# Autodesk Inventor assembly: ASY DMF 01 50 tape v2.1
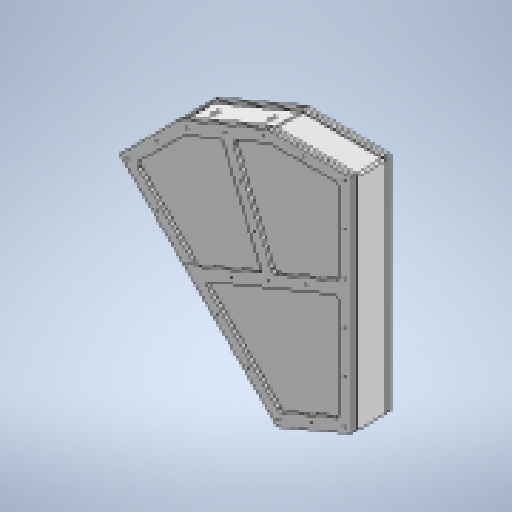
[picture p0: Inventor's stored thumbnail of the model, 512x512]
Saved by Autodesk Inventor 2025.3 (Build 293356000, 356)
## iProperties
Created: 2024-05-05
Part Number: ASY DMF 01 50 tape v2.1
Document SubType Name: Assembly
Designer: pokla
Author: pokla
## Documents named in this file (14)
- C:\Users\admin\Yandex.Disk\home pc\Inventor\DMF-Disk-Micro-Filter\Барабан v2.1\ASY DMF 01 50 tape v2.1.iam
- C:\Users\admin\Yandex.Disk\home pc\Inventor\DMF-Disk-Micro-Filter\Барабан v2.1\DMF 01 51 outside frame v2.1.ipt
- ДМС 201 Внешняя рамка.ipt
- C:\Users\admin\Yandex.Disk\home pc\Inventor\DMF-Disk-Micro-Filter\Барабан v2.1\DMF 01 52 Top sheet v2.1.ipt
- C:\Users\admin\Yandex.Disk\home pc\Inventor\DMF-Disk-Micro-Filter\Барабан v2.1\DMF 01 53 side part v2.1.ipt
- C:\Users\admin\Yandex.Disk\home pc\Inventor\DMF-Disk-Micro-Filter\Барабан v2.1\DMF 01 54 lower sheet v2.1.ipt
- C:\Users\admin\Yandex.Disk\home pc\Inventor\DMF-Disk-Micro-Filter\Барабан v2.1\DMF 01 56 Крепление сетки к кассете v2.1.ipt
- ДМС 206 Крепление сетки к кассете.ipt
- C:\Users\admin\Yandex.Disk\home pc\Inventor\DMF-Disk-Micro-Filter\Барабан v2.1\DMF 01 57 Сетка кассеты v2.1.ipt
- ДМС 207 Сетка кассеты.ipt
- C:\Users\admin\Yandex.Disk\home pc\Inventor\DMF-Disk-Micro-Filter\Барабан v2.1\DMF 01 51 outside frame_MIR1 v2.1.ipt
- C:\Users\admin\Yandex.Disk\home pc\Inventor\DMF-Disk-Micro-Filter\Барабан v2.1\DMF 01 56 Крепление сетки к кассете_MIR1 v2.1.ipt
- C:\Users\admin\Yandex.Disk\home pc\Inventor\DMF-Disk-Micro-Filter\Барабан v2.1\DMF 01 57 Сетка кассеты_MIR1 v2.1.ipt
- C:\Users\admin\Yandex.Disk\home pc\Inventor\DMF-Disk-Micro-Filter\Барабан v2.1\DMF 01 58 Фиксатор расстояния кассет v2.1.ipt
## Components (11 placed, 10 different names)
1. DMF 01 51 outside frame v2.1.ipt:1
2. DMF 01 52 Top sheet v2.1.ipt:1
3. DMF 01 53 side part v2.1.ipt:1
4. DMF 01 54 lower sheet v2.1.ipt:1
5. DMF 01 56 Крепление сетки к кассете v2.1.ipt:1
6. DMF 01 57 Сетка кассеты v2.1.ipt:1
7. DMF 01 53 side part v2.1.ipt:2
8. DMF 01 51 outside frame_MIR1 v2.1.ipt:1
9. DMF 01 56 Крепление сетки к кассете_MIR1 v2.1.ipt:1
10. DMF 01 57 Сетка кассеты_MIR1 v2.1.ipt:1
11. DMF 01 58 Фиксатор расстояния кассет v2.1.ipt:1
## Relationships (11: WeldJoint 7, RevoluteJoint 2, Mate 2)
- [WeldJoint]: DMF 01 51 outside frame v2.1.ipt:1 ↔ DMF 01 57 Сетка кассеты v2.1.ipt:1
- [WeldJoint]: DMF 01 51 outside frame v2.1.ipt:1 ↔ DMF 01 52 Top sheet v2.1.ipt:1
- [RevoluteJoint]: DMF 01 51 outside frame v2.1.ipt:1 ↔ DMF 01 53 side part v2.1.ipt:1
- [Mate]: DMF 01 51 outside frame v2.1.ipt:1 ↔ DMF 01 53 side part v2.1.ipt:1
- [WeldJoint] (0.5 mm): DMF 01 51 outside frame v2.1.ipt:1 ↔ DMF 01 56 Крепление сетки к кассете v2.1.ipt:1
- [RevoluteJoint]: DMF 01 51 outside frame v2.1.ipt:1 ↔ DMF 01 53 side part v2.1.ipt:2
- [Mate]: DMF 01 51 outside frame v2.1.ipt:1 ↔ DMF 01 53 side part v2.1.ipt:2
- [WeldJoint]: DMF 01 51 outside frame v2.1.ipt:1 ↔ DMF 01 54 lower sheet v2.1.ipt:1
- [WeldJoint] (0.5 mm): DMF 01 51 outside frame_MIR1 v2.1.ipt:1 ↔ DMF 01 56 Крепление сетки к кассете_MIR1 v2.1.ipt:1
- [WeldJoint]: DMF 01 51 outside frame_MIR1 v2.1.ipt:1 ↔ DMF 01 57 Сетка кассеты_MIR1 v2.1.ipt:1
- [WeldJoint]: DMF 01 52 Top sheet v2.1.ipt:1 ↔ DMF 01 58 Фиксатор расстояния кассет v2.1.ipt:1
## Named parameters: d0_d1 = 0 mm, d1_d3 = 0 mm, d2_d4 = 0 mm, d3_d5 = 90 deg, d4_d6 = 0 mm, d5_d7 = 0.5 mm, d6_d8 = 0 mm, d7_d9 = -90 deg, d8_d10 = 0 mm, d9_d11 = 0 mm
